# Autodesk Inventor assembly: Assembly
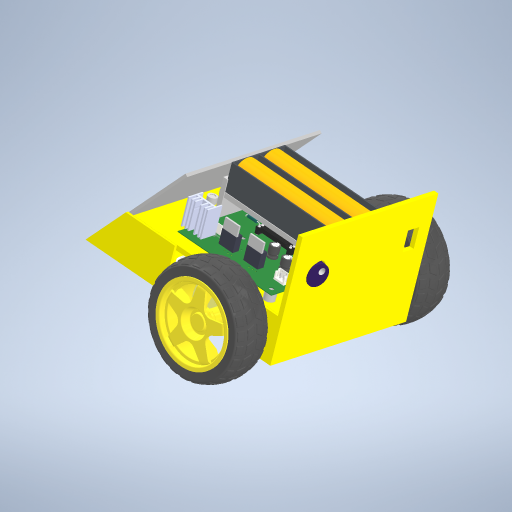
[picture p0: Inventor's stored thumbnail of the model, 512x512]
Saved by Autodesk Inventor 2024 (Build 280153000, 153)
## iProperties
Created: 2024-04-22
Part Number: Assembly
Document SubType Name: Assembly
Designer: samue
Author: samue
## Documents named in this file (14)
- D:\samue\Escritorio\OneDrive - UVG\UVG\Año 2024\Semestre 1\SIMULACION Y PCB\Altium\Sumo\Inventor\Assembly.iam
- D:\samue\Escritorio\OneDrive - UVG\UVG\Año 2024\Semestre 1\SIMULACION Y PCB\Altium\Sumo\Inventor\Base.ipt
- D:\samue\Escritorio\OneDrive - UVG\UVG\Año 2024\Semestre 1\SIMULACION Y PCB\Altium\Sumo\Inventor\MotoReductor.ipt
- D:\samue\Escritorio\OneDrive - UVG\UVG\Año 2024\Semestre 1\SIMULACION Y PCB\Altium\Sumo\Inventor\Yellow Motor Wheel\Yellow Motor Wheel.iam
- D:\samue\Escritorio\OneDrive - UVG\UVG\Año 2024\Semestre 1\SIMULACION Y PCB\Altium\Sumo\Inventor\Sujeta_motor.ipt
- D:\samue\Escritorio\OneDrive - UVG\UVG\Año 2024\Semestre 1\SIMULACION Y PCB\Altium\Sumo\Inventor\M4 x10.ipt
- D:\samue\Escritorio\OneDrive - UVG\UVG\Año 2024\Semestre 1\SIMULACION Y PCB\Altium\Sumo\Inventor\Empuja.ipt
- D:\samue\Escritorio\OneDrive - UVG\UVG\Año 2024\Semestre 1\SIMULACION Y PCB\Altium\Sumo\Inventor\PCB1\PCB1.ipt
- D:\samue\Escritorio\OneDrive - UVG\UVG\Año 2024\Semestre 1\SIMULACION Y PCB\Altium\Sumo\Inventor\Bateria\Bateria.ipt
- D:\samue\Escritorio\OneDrive - UVG\UVG\Año 2024\Semestre 1\SIMULACION Y PCB\Altium\Sumo\Inventor\Sos PCB.ipt
- D:\samue\Escritorio\OneDrive - UVG\UVG\Año 2024\Semestre 1\SIMULACION Y PCB\Altium\Sumo\Inventor\bate2.ipt
- D:\samue\Escritorio\OneDrive - UVG\UVG\Año 2024\Semestre 1\SIMULACION Y PCB\Altium\Sumo\Inventor\tapabate.ipt
- D:\samue\Escritorio\OneDrive - UVG\UVG\Año 2024\Semestre 1\SIMULACION Y PCB\Altium\Sumo\Inventor\PARED.ipt
- D:\samue\Escritorio\OneDrive - UVG\UVG\Año 2024\Semestre 1\SIMULACION Y PCB\Altium\Sumo\Inventor\Conector de carga.ipt
## Components (20 placed, 13 different names)
1. Base:1 — Mate:9, Mate:11, Mate:12, Mate:13, Mate:14, Mate:15, Mate:18, Mate:22, Mate:23, Mate:24, Mate:25, Mate:26, Mate:27, Mate:28, Mate:55, Mate:56, Mate:57, Mate:58, Mate:59, Mate:60
2. MotoReductor:1 — Rotational:1, Mate:15, Mate:16, Mate:17
3. MotoReductor:2 — Rotational:2, Mate:9, Mate:18, Mate:19
4. Yellow Motor Wheel:1 [sub-assembly] — Rotational:1
5. Yellow Motor Wheel:2 [sub-assembly] — Rotational:2
6. Sujeta_motor:1 — Mate:16, Mate:17, Mate:19, Mate:22, Mate:23, Mate:24, Mate:63
7. M4 x10:1 — Mate:11, Mate:12
8. M4 x10:2 — Mate:13, Mate:14
9. Empuja:1 — Mate:63
10. Bateria:1 — Mate:46, Flush:1
11. Sos PCB:1 — Mate:25, Mate:51, Mate:52
12. Sos PCB:2 — Mate:26, Mate:54
13. Sos PCB:3 — Mate:27, Mate:53
14. Sos PCB:4 — Mate:28, Mate:50
15. bate2:1 — Mate:58, Mate:59, Mate:60, Mate:61, Mate:62
16. bate2:2 — Mate:55, Mate:56, Mate:57
17. tapabate:1 — Mate:46, Flush:1, Mate:61, Mate:62
18. PCB1:1 — Mate:50, Mate:51, Mate:52, Mate:53, Mate:54
19. PARED:1
20. Conector de carga:1
## Relationships (35: Mate 32, RevoluteJoint 2, Flush 1)
- Rotational:1 [RevoluteJoint] (-7 mm): MotoReductor:1 ↔ Yellow Motor Wheel:1
- Rotational:2 [RevoluteJoint] (7 mm): MotoReductor:2 ↔ Yellow Motor Wheel:2
- Mate:9: Base:1 ↔ MotoReductor:2
- Mate:11: Base:1 ↔ M4 x10:1
- Mate:12: Base:1 ↔ M4 x10:1
- Mate:13: Base:1 ↔ M4 x10:2
- Mate:14: Base:1 ↔ M4 x10:2
- Mate:15: Base:1 ↔ MotoReductor:1
- Mate:16: MotoReductor:1 ↔ Sujeta_motor:1
- Mate:17: MotoReductor:1 ↔ Sujeta_motor:1
- Mate:18: Base:1 ↔ MotoReductor:2
- Mate:19: MotoReductor:2 ↔ Sujeta_motor:1
- Mate:22: Base:1 ↔ Sujeta_motor:1
- Mate:23: Base:1 ↔ Sujeta_motor:1
- Mate:24: Base:1 ↔ Sujeta_motor:1
- Mate:25: Base:1 ↔ Sos PCB:1
- Mate:26: Base:1 ↔ Sos PCB:2
- Mate:27: Base:1 ↔ Sos PCB:3
- Mate:28: Base:1 ↔ Sos PCB:4
- Mate:46: Bateria:1 ↔ tapabate:1
- Flush:1: Bateria:1 ↔ tapabate:1
- Mate:50: Sos PCB:4 ↔ PCB1:1
- Mate:51: Sos PCB:1 ↔ PCB1:1
- Mate:52: Sos PCB:1 ↔ PCB1:1
- Mate:53: Sos PCB:3 ↔ PCB1:1
- Mate:54: Sos PCB:2 ↔ PCB1:1
- Mate:55: Base:1 ↔ bate2:2
- Mate:56: Base:1 ↔ bate2:2
- Mate:57 (0.01 mm): Base:1 ↔ bate2:2
- Mate:58: Base:1 ↔ bate2:1
- Mate:59 (0.01 mm): Base:1 ↔ bate2:1
- Mate:60: Base:1 ↔ bate2:1
- Mate:61: bate2:1 ↔ tapabate:1
- Mate:62: bate2:1 ↔ tapabate:1
- Mate:63: Sujeta_motor:1 ↔ Empuja:1
